# Autodesk Inventor assembly: nc_nhk6
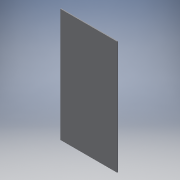
[picture p0: Inventor's stored thumbnail of the model, 180x180]
Saved by Autodesk Inventor 2019 (Build 230136000, 136)
## iProperties
Created: 2022-02-27
Part Number: nc_nhk6
Material: 一般
Document SubType Name: Assembly
Designer: yuta
Author: yuta
## Documents named in this file (5)
- C:\Users\yuta\Documents\NHK\nc_nhk6.iam
- C:\Users\yuta\Documents\NHK\NC.1.ipt
- C:\Users\yuta\Documents\NHK\nhk46.ipt
- C:\Users\yuta\Documents\NHK\nhk45.ipt
- C:\Users\yuta\Documents\NHK\nhk47.ipt
## Components (4 placed, 4 different names)
1. NC.1:1 — メイト:1, メイト:2, メイト:3
2. nhk46:1 — メイト:1
3. nhk45:1 — メイト:2
4. nhk47:1 — メイト:3
## Relationships (3: Mate 3)
- メイト:1 [Mate]: NC.1:1 ↔ nhk46:1
- メイト:2 [Mate]: NC.1:1 ↔ nhk45:1
- メイト:3 [Mate]: NC.1:1 ↔ nhk47:1
